# Autodesk Inventor assembly: Assembly
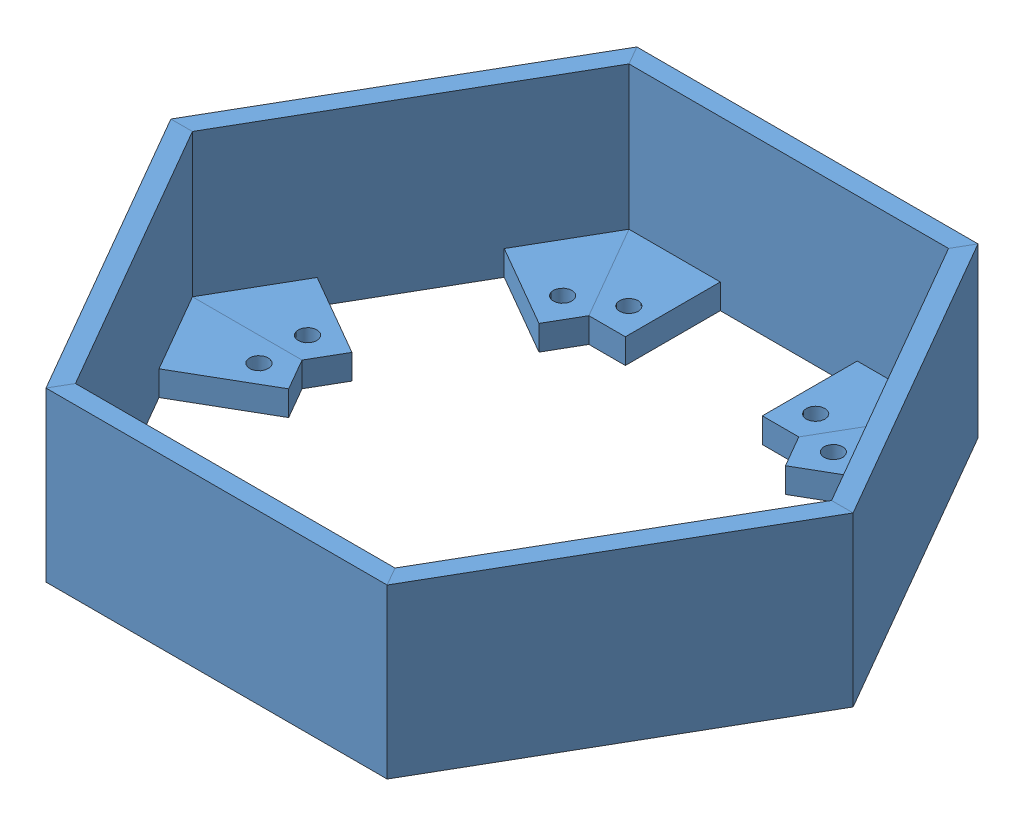
[picture p0: shaded view drawn from the shape stored in the file]
Saved by Autodesk Inventor 2018 (Build 220112000, 112)
## iProperties
Created: 2017-04-19
Part Number: Assembly
Document SubType Name: Assembly
Designer: Pablo
Author: Pablo
## Documents named in this file (2)
- C:\Users\Pablo\Desktop\Assembly.iam
- J:\mp3mp3.ipt
## Components (6 placed, 1 different names)
1. mp3mp3:1 — Mate:1, Flush:1, Flush:2, Flush:3, Flush:4, Flush:5, Mate:6, Mate:7
2. mp3mp3:2 — Mate:1, Flush:1, Mate:2, Mate:7, Mate:8
3. mp3mp3:3 — Flush:4, Mate:4, Mate:5, Mate:10
4. mp3mp3:4 — Mate:2, Flush:2, Mate:3, Mate:8, Mate:9
5. mp3mp3:5 — Flush:3, Mate:5, Mate:6
6. mp3mp3:6 — Flush:5, Mate:3, Mate:4, Mate:9, Mate:10
## Relationships (15: Mate 10, Flush 5)
- Mate:1: mp3mp3:1 ↔ mp3mp3:2
- Flush:1: mp3mp3:1 ↔ mp3mp3:2
- Mate:2: mp3mp3:2 ↔ mp3mp3:4
- Flush:2: mp3mp3:1 ↔ mp3mp3:4
- Flush:3: mp3mp3:1 ↔ mp3mp3:5
- Flush:4: mp3mp3:1 ↔ mp3mp3:3
- Flush:5: mp3mp3:1 ↔ mp3mp3:6
- Mate:3: mp3mp3:4 ↔ mp3mp3:6
- Mate:4: mp3mp3:3 ↔ mp3mp3:6
- Mate:5: mp3mp3:3 ↔ mp3mp3:5
- Mate:6: mp3mp3:1 ↔ mp3mp3:5
- Mate:7: mp3mp3:1 ↔ mp3mp3:2
- Mate:8: mp3mp3:2 ↔ mp3mp3:4
- Mate:9: mp3mp3:4 ↔ mp3mp3:6
- Mate:10: mp3mp3:3 ↔ mp3mp3:6
